# Autodesk Inventor assembly: Retro PC
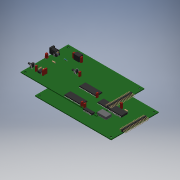
[picture p0: Inventor's stored thumbnail of the model, 180x180]
Saved by Autodesk Inventor 2019 (Build 230136000, 136)
## iProperties
Created: 2019-12-02
Part Number: Retro PC
Material: Generisch
Document SubType Name: Assembly
Designer: Daniel
Author: Daniel
## Documents named in this file (3)
- G:\Dropbox\Git\Retro PC\drawing\Retro PC.iam
- G:\Dropbox\Git\Retro PC\export\PowerSupply.ipt
- G:\Dropbox\Git\Retro PC\export\ProcessorBoardProcessorBoard.ipt
## Components (2 placed, 2 different names)
1. PowerSupply:1 — Passend:1
2. ProcessorBoardProcessorBoard:1 — Passend:1
## Relationships (1: Mate 1)
- Passend:1 [Mate]: PowerSupply:1 ↔ ProcessorBoardProcessorBoard:1
